# Autodesk Inventor assembly: Bottom_Foot_Assembly
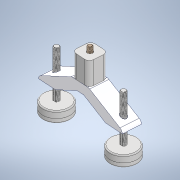
[picture p0: Inventor's stored thumbnail of the model, 180x180]
Saved by Autodesk Inventor 2021 (Build 250183000, 183)
## iProperties
Created: 2022-01-01
Part Number: Bottom_Foot_Assembly
Document SubType Name: Assembly
Designer: Jorian Bruslind
Author: Jorian Bruslind
## Documents named in this file (6)
- C:\Users\Jorian Bruslind\Documents\GitHub\PersonalProjects\HyperRail\Inventor Files\Bottom_Foot_Assembly.iam
- C:\Users\Jorian Bruslind\Documents\GitHub\PersonalProjects\HyperRail\Inventor Files\Bottom_Foot_Standoff.ipt
- C:\Users\Jorian Bruslind\Documents\GitHub\PersonalProjects\HyperRail\Inventor Files\SpacerBlock_25mm.ipt
- C:\Users\Jorian Bruslind\Documents\GitHub\PersonalProjects\HyperRail\Inventor Files\McMaster Files\Leveling Feet\62805K49_Heavy Duty Leveling Mount.ipt
- C:\Users\Jorian Bruslind\Documents\GitHub\PersonalProjects\HyperRail\Inventor Files\Metric bolt\Bolt M5 40mm.ipt
- C:\Users\Jorian Bruslind\Documents\GitHub\PersonalProjects\HyperRail\Inventor Files\Metric nuts\Nut M6.ipt
## Components (7 placed, 5 different names)
1. Bottom_Foot_Standoff:1 — Angle:1, Flush:3, Angle:2, Flush:4
2. SpacerBlock_25mm:1
3. 62805K49_Heavy Duty Leveling Mount:1 — Mate:8
4. 62805K49_Heavy Duty Leveling Mount:2 — Mate:9
5. Bolt M5 40mm:1
6. Nut M6:1 — Mate:9, Angle:2, Flush:4
7. Nut M6:2 — Mate:8, Angle:1, Flush:3
## Relationships (15: Mate 9, Flush 4, Angle 2)
- [Mate]: Bottom_Foot_Standoff:1 ↔ SpacerBlock_25mm:1
- [Mate]: Bottom_Foot_Standoff:1 ↔ SpacerBlock_25mm:1
- [Flush]: Bottom_Foot_Standoff:1 ↔ SpacerBlock_25mm:1
- [Mate]: Bottom_Foot_Standoff:1 ↔ 62805K49_Heavy Duty Leveling Mount:1
- [Mate]: Bottom_Foot_Standoff:1 ↔ 62805K49_Heavy Duty Leveling Mount:2
- [Flush]: 62805K49_Heavy Duty Leveling Mount:1 ↔ 62805K49_Heavy Duty Leveling Mount:2
- [Mate] (20 mm): Bottom_Foot_Standoff:1 ↔ 62805K49_Heavy Duty Leveling Mount:1
- [Mate]: Bottom_Foot_Standoff:1 ↔ Bolt M5 40mm:1
- [Mate]: Bottom_Foot_Standoff:1 ↔ Bolt M5 40mm:1
- Mate:8: 62805K49_Heavy Duty Leveling Mount:1 ↔ Nut M6:2
- Angle:1 (0 deg): Bottom_Foot_Standoff:1 ↔ Nut M6:2
- Flush:3: Bottom_Foot_Standoff:1 ↔ Nut M6:2
- Mate:9: 62805K49_Heavy Duty Leveling Mount:2 ↔ Nut M6:1
- Angle:2 (0 deg): Bottom_Foot_Standoff:1 ↔ Nut M6:1
- Flush:4: Bottom_Foot_Standoff:1 ↔ Nut M6:1
## Named parameters: d770_d759 = 0 mm, d771_d760 = 0 mm, d772_d761 = 0 mm, d773_d762 = 20 mm, d774_d752 = 0 mm, d775_d753 = 0 mm, d776_d754 = 0 mm
